# Autodesk Inventor assembly: leg2
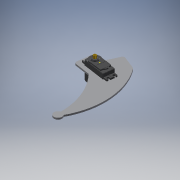
[picture p0: Inventor's stored thumbnail of the model, 180x180]
Saved by Autodesk Inventor 2019 (Build 230136000, 136)
## iProperties
Created: 2023-04-16
Part Number: leg2
Document SubType Name: Assembly
Designer: Analuam
Author: Analuam
## Documents named in this file (3)
- D:\Dek Diyah\leg2.iam
- D:\Dek Diyah\Part3.ipt
- D:\Dek Diyah\Servo berputar.iam
## Components (2 placed, 2 different names)
1. Servo berputar:4 [sub-assembly] — Mate:13, Mate:14, Mate:15
2. Part3:4 — Mate:13, Mate:14, Mate:15
## Relationships (3: Mate 3)
- Mate:13: Servo berputar:4 ↔ Part3:4
- Mate:14: Servo berputar:4 ↔ Part3:4
- Mate:15: Servo berputar:4 ↔ Part3:4
